# Autodesk Inventor assembly: temporary
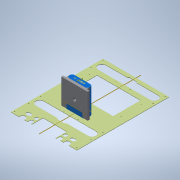
[picture p0: Inventor's stored thumbnail of the model, 180x180]
Saved by Autodesk Inventor 2020.2 (Build 242310000, 310)
## iProperties
Created: 2020-09-24
Part Number: temporary
Material: 一般
Document SubType Name: Assembly
Designer: gisen
Author: gisen
## Documents named in this file (3)
- C:\Users\gisen\GitProjects\CAD-Data\CuboidSubcomponents\temporary.iam
- C:\Users\gisen\GitProjects\CAD-Data\CuboidSubcomponents\out_front.ipt
- C:\Users\gisen\GitProjects\CAD-Data\AzureKinect\AzureKinectAssembly.iam
## Components (2 placed, 2 different names)
1. out_front:1 — フラッシュ:1, メイト:1, メイト:2
2. AzureKinectAssembly:1 [sub-assembly] — フラッシュ:1, メイト:1, メイト:2
## Relationships (3: Mate 2, Flush 1)
- フラッシュ:1 [Flush]: out_front:1 ↔ AzureKinectAssembly:1
- メイト:1 [Mate]: out_front:1 ↔ AzureKinectAssembly:1
- メイト:2 [Mate]: out_front:1 ↔ AzureKinectAssembly:1
